# Autodesk Inventor assembly: EFOI-10
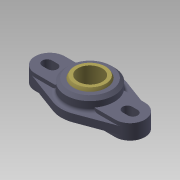
[picture p0: Inventor's stored thumbnail of the model, 180x180]
Saved by Autodesk Inventor 2020.1 (Build 241239000, 239)
## iProperties
Created: 2019-12-11
Part Number: EFOI-10
Document SubType Name: Assembly
Project: FIRST
Catalog Web Link: http://www.igus.com/wpck/5378/igubal_Flanschlager_EFOI?CL=US-en
Description: Flanged spherical bearing
Vendor: igus
Category: FIRST 2020 KOP
Company: Autodesk, Inc.
Title: Flanged Spherical Bearing
Author: Autodesk, Inc.
## Documents named in this file (3)
- D:\FIRST 2020\FRC 2020\FRC KOP 2020\Inventor\EFOI-10R.iam
- D:\FIRST 2020\FRC 2020\FRC KOP 2020\Inventor\Parts\EFOI-10_Housing.ipt
- D:\FIRST 2020\FRC 2020\FRC KOP 2020\Inventor\Parts\EFOI-10_Spherical Bearing.ipt
## Components (2 placed, 2 different names)
1. EFOI-10_Housing:1 — Mate:1
2. EFOI-10_Spherical Bearing:1 — Mate:1
## Relationships (1: Mate 1)
- Mate:1: EFOI-10_Housing:1 ↔ EFOI-10_Spherical Bearing:1
